# Autodesk Inventor assembly: SBGTN6900VV
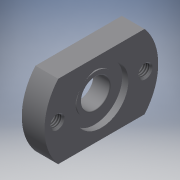
[picture p0: Inventor's stored thumbnail of the model, 180x180]
Saved by Autodesk Inventor 2019 (Build 230136000, 136)
## iProperties
Category: PARTsolutions
Company: MISUMI
Created: 2022-11-14
Part Number: SBGTN6900VV
Catalog Web Link: www.cadenas.de
Description: BGTNB, BGTN, SBGTN-Bearings with Housings - Space Saving, Small Flange - Non-Retained
Vendor: MISUMI
Document SubType Name: Assembly
Designer: psAdmin
Manufacturer: MISUMI
Mass: 6.2831 g
Surface Area: 42.4439 cm^2
Volume: 6.2831 cm^3
Density: 1 g/cm^3
Title: SBGTN6900VV
Author: Cadenas PARTsolutions
Comments: Bearings with Housings - Space Saving, Small Flange - Non-Retained
PSOL_IDENT_0: {$CADENAS_DATA/23d-libs/misumi/metric/12_bearing_holders/bgtnb_asmtab.prj},205 {VTYP=3D},{STYP=ASSTA
PSOL_IDENT_1: B},{NB=SBGTN6900VV},{LINA=SBGTN6900VV},{NN=BGTNB, BGTN, SBGTN},{DATE=30.06.2021 12:58:21},{GEOMDATE=
PSOL_IDENT_2: 10.07.2015 02:16:54},{VERSION=},{LINEID=90},{WBVAR=MATB,ST,SEAL,ALT1},{WBNUMERIC=}  {NB=SBGTN6900VV}
PSOL_IDENT_3: ,{LINA=SBGTN6900VV},{KT=DUMMY},{PN=SBGTN6900VV},{TYPE=SBGTN},{MATB=SS},{MATBALG= 'S' , 'Steel' , 'SS'
PSOL_IDENT_4: , 'Stainless Steel' },{ST=-},{STALG= '-' , '-' },{BN=6900},{SEAL=VV},{SEALALG= 'ZZ' , 'Double Shiel
PSOL_IDENT_5: ded' , 'VV' , 'Non-Contact Sealed Rubber Seal' , 'DD' , 'Contact Sealed Rubber Seal' },{DD=10},{D=22
PSOL_IDENT_6: },{B=6},{H=40},{W=26},{T=8},{DDHH=19},{A=31},{F=0},{M=M5},{ALT1=},{M3D=5},{PPATH=bgtnb/bgtnb_asmtpl.
PSOL_IDENT_7: prj}
NB: SBGTN6900VV
NN: BGTNB, BGTN, SBGTN
NT: Bearings with Housings - Space Saving, Small Flange - Non-Retained
NBSYN: $PN.
LINA: SBGTN6900VV
CATALOG: Misumi
PN: SBGTN6900VV
MATB: Stainless Steel
ST: -
BN: 6900
SEAL: Non-Contact Sealed Rubber Seal
DD: 10
D: 22
B: 6
H: 40
W: 26
T: 8
DDHH: 19
A: 31
F: 0
M: M5
ALT1: Bearing and Retaining Ring Assembled
SUPPLIER: MISUMI
ARTICLENO: SBGTN6900VV
BOMINFO: SBGTN6900VV
CREATOR: CADENAS GmbH
## Documents named in this file (3)
- e:\temp\worker_COMMON_2\temp\tmp_7512_18_p0Bxq\format_0\SBGTN6900VV.iam
- e:\temp\worker_COMMON_2\temp\tmp_7512_18_p0Bxq\format_0\SBGTN6900VV_h.ipt
- e:\temp\worker_COMMON_2\temp\tmp_7512_18_p0Bxq\format_0\bearing_6900.ipt
## Components (2 placed, 2 different names)
1. SBGTN6900VV_h:1 — to_bearings_XY@1 <-> to_housing_XY@2, to_bearings_Z@1 <-> to_housing_Z@2, to_bearings_YZ@1 <-> to_housing_YZ@2
2. bearing_6900:1 — to_bearings_XY@1 <-> to_housing_XY@2, to_bearings_Z@1 <-> to_housing_Z@2, to_bearings_YZ@1 <-> to_housing_YZ@2
## Relationships (3: Mate 2, Angle 1)
- to_bearings_XY@1 <-> to_housing_XY@2 [Mate]: SBGTN6900VV_h:1 ↔ bearing_6900:1
- to_bearings_Z@1 <-> to_housing_Z@2 [Mate]: SBGTN6900VV_h:1 ↔ bearing_6900:1
- to_bearings_YZ@1 <-> to_housing_YZ@2 [Angle] (0 deg): SBGTN6900VV_h:1 ↔ bearing_6900:1
